# Autodesk Inventor assembly: ADL5534-Enclosure
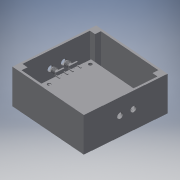
[picture p0: Inventor's stored thumbnail of the model, 180x180]
Saved by Autodesk Inventor 2018 (Build 220112000, 112)
## iProperties
Created: 2018-04-27
Part Number: ADL5534-Enclosure
Document SubType Name: Assembly
Designer: bbramman
Author: bbramman
## Documents named in this file (4)
- C:\Users\bbramman\OneDrive\Documents\Trapped Ion Research (Grad)\Electronics\pll-evalboard-synthesizer\Box CAD\ADL5534-Enclosure.iam
- C:\Users\bbramman\OneDrive\Documents\Trapped Ion Research (Grad)\Electronics\pll-evalboard-synthesizer\Box CAD\546-1590YFLBK-ADL5534.ipt
- C:\Users\bbramman\OneDrive\Documents\Trapped Ion Research (Grad)\Electronics\pll-evalboard-synthesizer\Box CAD\EV-ADL5534.iam
- C:\Users\bbramman\OneDrive\Documents\Trapped Ion Research (Grad)\Electronics\pll-evalboard-synthesizer\Box CAD\Power-Reg.iam
## Components (3 placed, 3 different names)
1. EV-ADL5534:1 [sub-assembly] — Insert:3
2. Power-Reg:1 [sub-assembly] — Insert:2
3. 546-1590YFLBK-ADL5534:1 — Insert:2, Insert:3
## Relationships (2: Insert 2)
- Insert:2 (8.8392 mm): Power-Reg:1 ↔ 546-1590YFLBK-ADL5534:1
- Insert:3 (19.05 mm): EV-ADL5534:1 ↔ 546-1590YFLBK-ADL5534:1
